# Autodesk Inventor assembly: 3D HUMAN
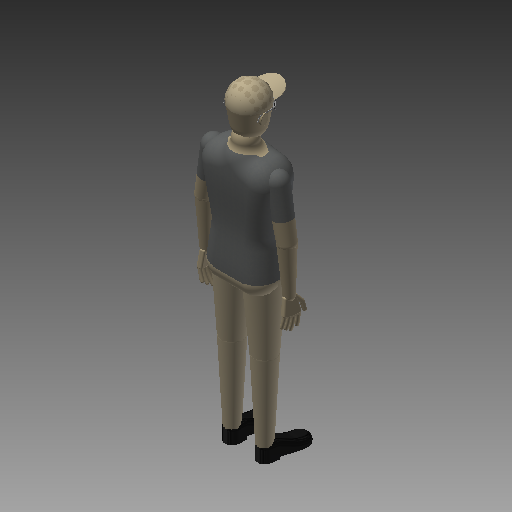
[picture p0: Inventor's stored thumbnail of the model, 512x512]
Saved by Autodesk Inventor 2019 (Build 230136000, 136)
## iProperties
Category: ASSY
Shininess: 64.0
Length Units: 11272
Angle Units: 11279
Time Units: 11290
Mass Units: 11286
Length Display Precision: 3
Angle Display Precision: 2
Compacted: True
Part Number: 3D HUMAN
Document SubType Name: Assembly
Created: 2003-03-22
Designer: M.F.
Catalog Web Link: www.apollocanard.com
Density: 0.0
Volumn: 0.0
Area: 0.0
PropertySet Name: Model Information
Control State: 0
Master: False
Checked Out: False
Title: iMan
Author: M.F.
## Documents named in this file (14)
- \\Mac\Home\Downloads\iManikins\iMan\iMan.iam
- \\Mac\Home\Downloads\iManikins\iMan\iMan - 2D BODY.ipt
- \\Mac\Home\Downloads\iManikins\iMan\iMan - HAT.ipt
- \\Mac\Home\Downloads\iManikins\iMan\iMan - HEAD.ipt
- \\Mac\Home\Downloads\iManikins\iMan\iMan - ARM UPPER.ipt
- \\Mac\Home\Downloads\iManikins\iMan\iMan - ARM LOWER.ipt
- \\Mac\Home\Downloads\iManikins\iMan\iMan - LEG UPPER.ipt
- \\Mac\Home\Downloads\iManikins\iMan\iMan - LEG LOWER.ipt
- \\Mac\Home\Downloads\iManikins\iMan\iMan - FOOT.ipt
- \\Mac\Home\Downloads\iManikins\iMan\iMan - HAND.ipt
- \\Mac\Home\Downloads\iManikins\iMan\iMan - FINGERS LEFT.ipt
- \\Mac\Home\Downloads\iManikins\iMan\iMan - FINGERS RIGHT.ipt
- \\Mac\Home\Downloads\iManikins\iMan\iMan - SHADES.ipt
- \\Mac\Home\Downloads\iManikins\iMan\iMan - TORSO.ipt
## Components (19 placed, 13 different names)
1. iMan - 2D BODY:1 — Flush:1, Flush:2, Flush:7
2. iMan - TORSO:1 — Flush:4, Flush:6, LEFT FOOT TWIST ANGLE, LEG STRADDLE DIST1, LEG STRADDLE DIST2, Flush:7, LEFT FOOT FLAT, RIGHT FOOT FLAT, Tangent:3, Mate:17, Mate:18
3. iMan - ARM UPPER:1 — Mate:1
4. iMan - ARM LOWER:1 — Mate:1, Mate:4
5. iMan - LEG UPPER:1 — Mate:2
6. iMan - LEG LOWER:1 — Mate:2, Mate:3, LEG STRADDLE DIST1, Tangent:1
7. iMan - FOOT:1 — Mate:3, LEFT FOOT TWIST ANGLE, Tangent:1, LEFT FOOT FLAT
8. iMan - HAND:1 — Mate:4, Mate:5, Mate:6, LEFT FINGERS CLOSED ANGLE
9. iMan - FINGERS LEFT:1 — Mate:5, Mate:6, LEFT FINGERS CLOSED ANGLE
10. iMan - ARM UPPER:2 — Mate:7
11. iMan - ARM LOWER:2 — Mate:7, Mate:10, Mate:11
12. iMan - LEG UPPER:2 — Mate:8
13. iMan - LEG LOWER:2 — Mate:8, Mate:9, LEG STRADDLE DIST2, Tangent:2
14. iMan - FOOT:2 — Mate:9, Tangent:2, RIGHT FOOT FLAT
15. iMan - HAND:2 — Mate:10, Mate:11, Flush:3, Mate:12, RIGHT FINGERS CLOSED ANGLE
16. iMan - FINGERS RIGHT:1 — Flush:3, Mate:12, RIGHT FINGERS CLOSED ANGLE
17. iMan - SHADES:1 — Tangent:4, Mate:20
18. iMan - HAT:1 — Mate:19
19. iMan - HEAD:1 — Tangent:3, Mate:17, Mate:18, Mate:19, Tangent:4, Mate:20
## Relationships (44: Mate 22, Flush 9, Angle 9, Tangent 4)
- Flush:1: iMan - 2D BODY:1
- Flush:2: iMan - 2D BODY:1
- Mate:1: iMan - ARM UPPER:1 ↔ iMan - ARM LOWER:1
- Mate:2: iMan - LEG UPPER:1 ↔ iMan - LEG LOWER:1
- Mate:3: iMan - LEG LOWER:1 ↔ iMan - FOOT:1
- Mate:4: iMan - ARM LOWER:1 ↔ iMan - HAND:1
- Mate:5: iMan - HAND:1 ↔ iMan - FINGERS LEFT:1
- Mate:6: iMan - HAND:1 ↔ iMan - FINGERS LEFT:1
- [Mate]: iMan - ARM LOWER:1 ↔ iMan - HAND:1
- LEFT FINGERS CLOSED ANGLE [Angle] (15 deg): iMan - HAND:1 ↔ iMan - FINGERS LEFT:1
- Mate:7: iMan - ARM UPPER:2 ↔ iMan - ARM LOWER:2
- Mate:8: iMan - LEG UPPER:2 ↔ iMan - LEG LOWER:2
- Mate:9: iMan - LEG LOWER:2 ↔ iMan - FOOT:2
- Mate:10: iMan - ARM LOWER:2 ↔ iMan - HAND:2
- Mate:11: iMan - ARM LOWER:2 ↔ iMan - HAND:2
- Flush:3: iMan - HAND:2 ↔ iMan - FINGERS RIGHT:1
- Mate:12: iMan - HAND:2 ↔ iMan - FINGERS RIGHT:1
- RIGHT FINGERS CLOSED ANGLE [Angle] (-15 deg): iMan - HAND:2 ↔ iMan - FINGERS RIGHT:1
- [Mate]: iMan - TORSO:1 ↔ iMan - ARM UPPER:1
- Flush:4: iMan - TORSO:1
- [Flush]: iMan - TORSO:1
- Flush:6: iMan - TORSO:1
- LEFT FOOT TWIST ANGLE [Angle] (5 deg): iMan - TORSO:1 ↔ iMan - FOOT:1
- [Mate]: iMan - TORSO:1 ↔ iMan - ARM UPPER:2
- LEG STRADDLE DIST1 [Flush] (88.9 mm): iMan - TORSO:1 ↔ iMan - LEG LOWER:1
- LEG STRADDLE DIST2 [Flush] (-88.9 mm): iMan - TORSO:1 ↔ iMan - LEG LOWER:2
- [Angle] (5 deg): iMan - TORSO:1 ↔ iMan - FOOT:2
- Flush:7: iMan - 2D BODY:1 ↔ iMan - TORSO:1
- [Mate]: iMan - TORSO:1 ↔ iMan - LEG UPPER:1
- [Mate]: iMan - TORSO:1 ↔ iMan - LEG UPPER:2
- Tangent:1: iMan - LEG LOWER:1 ↔ iMan - FOOT:1
- Tangent:2: iMan - LEG LOWER:2 ↔ iMan - FOOT:2
- LEFT FOOT FLAT [Angle] (180 deg): iMan - TORSO:1 ↔ iMan - FOOT:1
- RIGHT FOOT FLAT [Angle] (-180 deg): iMan - TORSO:1 ↔ iMan - FOOT:2
- Tangent:3: iMan - TORSO:1 ↔ iMan - HEAD:1
- Mate:17: iMan - TORSO:1 ↔ iMan - HEAD:1
- Mate:18 (20.32 mm): iMan - TORSO:1 ↔ iMan - HEAD:1
- Mate:19: iMan - HAT:1 ↔ iMan - HEAD:1
- Tangent:4: iMan - SHADES:1 ↔ iMan - HEAD:1
- Mate:20: iMan - SHADES:1 ↔ iMan - HEAD:1
- [Mate]: iMan - SHADES:1 ↔ iMan - HEAD:1
- [Angle] (3 deg): iMan - SHADES:1 ↔ iMan - HEAD:1
- [Angle] (0 deg): iMan - HAT:1 ↔ iMan - HEAD:1
- [Angle] (5 deg): iMan - HAT:1 ↔ iMan - HEAD:1
## Named parameters: LEG_STRADDLE_DIST_UNDER = 88.9 mm, LEFT_FINGERS_CLOSED_ANGLE = 15 deg, RIGHT_FINGERS_CLOSED_ANGLE = -15 deg
